# Autodesk Inventor assembly: X_rail_Assembly_Rev3
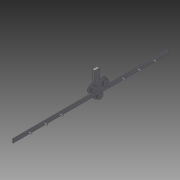
[picture p0: Inventor's stored thumbnail of the model, 180x180]
Saved by Autodesk Inventor 2015 (Build 190159000, 159)
## iProperties
Created: 2017-01-08
Part Number: X_rail_Assembly_Rev3
Document SubType Name: Assembly
Designer: Guy
Author: Guy
## Documents named in this file (5)
- C:\Users\Guy\Documents\Fourth Year\Capstone\git\Capstone-Project\doc\CAD\LowLevel_Rev3\X_rail_Assembly_Rev3.iam
- C:\Users\Guy\Documents\Fourth Year\Capstone\git\Capstone-Project\doc\CAD\LowLevel_Rev3\X_Rai-SquareBar-Rev3.ipt
- C:\Users\Guy\Documents\Fourth Year\Capstone\git\Capstone-Project\doc\CAD\LowLevel_Rev3\XY_Wheel-SquareBar-Rev3.ipt
- C:\Users\Guy\Documents\Fourth Year\Capstone\git\Capstone-Project\doc\CAD\LowLevel_Rev3\Arm_Base-SquareBar-Rev3.ipt
- C:\Users\Guy\Documents\Fourth Year\Capstone\git\Capstone-Project\doc\CAD\LowLevel_Rev3\Arm-SquareBar-Rev3.ipt
## Components (6 placed, 4 different names)
1. X_Rai-SquareBar-Rev3:1 — Tangent:1, Tangent:2, Tangent:3, Mate:1, Mate:2, Mate:3
2. XY_Wheel-SquareBar-Rev3:1 — Tangent:3, Mate:3, Mate:6
3. XY_Wheel-SquareBar-Rev3:2 — Tangent:2, Mate:2, Mate:5, Mate:7
4. XY_Wheel-SquareBar-Rev3:3 — Tangent:1, Mate:1, Mate:4
5. Arm_Base-SquareBar-Rev3:1 — Mate:4, Mate:5, Mate:6, Mate:7, Mate:8, Mate:9, Mate:10
6. Arm-SquareBar-Rev3:1 — Mate:8, Mate:9, Mate:10
## Relationships (13: Mate 10, Tangent 3)
- Tangent:1: X_Rai-SquareBar-Rev3:1 ↔ XY_Wheel-SquareBar-Rev3:3
- Tangent:2: X_Rai-SquareBar-Rev3:1 ↔ XY_Wheel-SquareBar-Rev3:2
- Tangent:3: X_Rai-SquareBar-Rev3:1 ↔ XY_Wheel-SquareBar-Rev3:1
- Mate:1 (0.5 mm): X_Rai-SquareBar-Rev3:1 ↔ XY_Wheel-SquareBar-Rev3:3
- Mate:2 (0.5 mm): X_Rai-SquareBar-Rev3:1 ↔ XY_Wheel-SquareBar-Rev3:2
- Mate:3 (0.5 mm): X_Rai-SquareBar-Rev3:1 ↔ XY_Wheel-SquareBar-Rev3:1
- Mate:4: XY_Wheel-SquareBar-Rev3:3 ↔ Arm_Base-SquareBar-Rev3:1
- Mate:5: XY_Wheel-SquareBar-Rev3:2 ↔ Arm_Base-SquareBar-Rev3:1
- Mate:6: XY_Wheel-SquareBar-Rev3:1 ↔ Arm_Base-SquareBar-Rev3:1
- Mate:7 (20 mm): XY_Wheel-SquareBar-Rev3:2 ↔ Arm_Base-SquareBar-Rev3:1
- Mate:8: Arm_Base-SquareBar-Rev3:1 ↔ Arm-SquareBar-Rev3:1
- Mate:9: Arm_Base-SquareBar-Rev3:1 ↔ Arm-SquareBar-Rev3:1
- Mate:10: Arm_Base-SquareBar-Rev3:1 ↔ Arm-SquareBar-Rev3:1
